# Autodesk Inventor assembly: universal joint
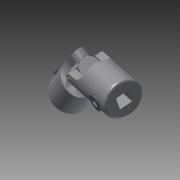
[picture p0: Inventor's stored thumbnail of the model, 180x180]
Saved by Autodesk Inventor 2015 SP1 (Build 190203100, 203)
## iProperties
Created: 2015-09-27
Part Number: universal joint
Document SubType Name: Assembly
Designer: Christopher
Title: 276-2045-002-000 Rev2.STEP
Description: STEP AP203
Creation Date: 2012-02-01
Sending System: SolidWorks 2011
Preprocessor: SwSTEP 2.0
Author: Christopher
## Documents named in this file (5)
- F:\VEX CAD Library\Motion\Universal Joint.iam
- F:\VEX CAD Library\Motion\Universal Joint Axle.ipt
- F:\VEX CAD Library\Motion\Universal Joint Set Screw.ipt
- F:\VEX CAD Library\Motion\Universal Joint Hub.ipt
- F:\VEX CAD Library\Motion\Universal Joint Link.ipt
## Components (7 placed, 7 different names)
1. 276-2045-002-003 Rev1_1 — Mate:2, Mate:4, Mate:6, Mate:9
2. 276-2045-002-004 Rev1_2 — Mate:8, Flush:2
3. 276-2045-002-002 Rev2_3 — Mate:3, Mate:4, Mate:9, Mate:10
4. 276-2045-002-004 Rev1_4 — Mate:1, Flush:1
5. 276-2045-002-001 Rev1_5 — Mate:5, Mate:7, Mate:8, Flush:2
6. 276-2045-002-003 Rev1_6 — Mate:3, Mate:5, Mate:7, Mate:10
7. 276-2045-002-001 Rev1_7 — Mate:1, Mate:2, Flush:1, Mate:6
## Relationships (12: Mate 10, Flush 2)
- Mate:1: 276-2045-002-004 Rev1_4 ↔ 276-2045-002-001 Rev1_7
- Mate:2: 276-2045-002-003 Rev1_1 ↔ 276-2045-002-001 Rev1_7
- Flush:1: 276-2045-002-004 Rev1_4 ↔ 276-2045-002-001 Rev1_7
- Mate:3: 276-2045-002-002 Rev2_3 ↔ 276-2045-002-003 Rev1_6
- Mate:4: 276-2045-002-003 Rev1_1 ↔ 276-2045-002-002 Rev2_3
- Mate:5: 276-2045-002-001 Rev1_5 ↔ 276-2045-002-003 Rev1_6
- Mate:6: 276-2045-002-003 Rev1_1 ↔ 276-2045-002-001 Rev1_7
- Mate:7: 276-2045-002-001 Rev1_5 ↔ 276-2045-002-003 Rev1_6
- Mate:8: 276-2045-002-004 Rev1_2 ↔ 276-2045-002-001 Rev1_5
- Flush:2: 276-2045-002-004 Rev1_2 ↔ 276-2045-002-001 Rev1_5
- Mate:9: 276-2045-002-003 Rev1_1 ↔ 276-2045-002-002 Rev2_3
- Mate:10: 276-2045-002-002 Rev2_3 ↔ 276-2045-002-003 Rev1_6
